# Autodesk Inventor assembly: ASY MSC 400 Accsess hatch
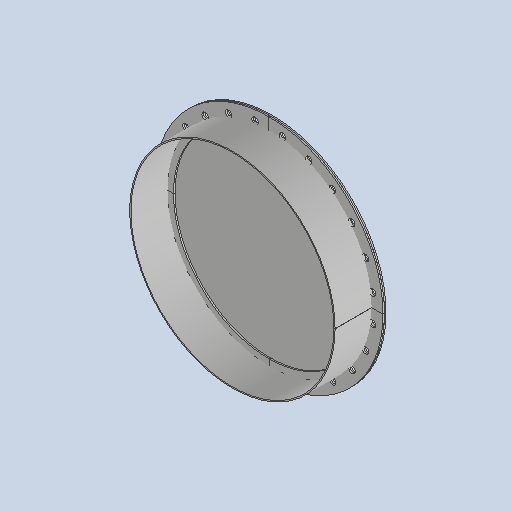
[picture p0: Inventor's stored thumbnail of the model, 512x512]
Saved by Autodesk Inventor 2025 (Build 290162010, 162A)
## iProperties
Created: 2024-09-04
Part Number: ASY MSC 400 Accsess hatch
Document SubType Name: Assembly
Designer: admin
Stock Number: ASY МОО 400 люк доступа
Author: admin
## Documents named in this file (6)
- C:\Users\DELL\YandexDisk-badmisterfox\домашниий пк\Inventor\Manturovo\Manturovo_Se-clar\ASY MSC 400 Accsess hatch.iam
- C:\Users\DELL\YandexDisk-badmisterfox\домашниий пк\Inventor\Manturovo\Manturovo_Se-clar\MSC 402 ring.ipt
- C:\Users\DELL\YandexDisk-badmisterfox\домашниий пк\Inventor\Manturovo\Manturovo_Se-clar\MSC 403 flange 500.ipt
- C:\Users\DELL\YandexDisk-badmisterfox\домашниий пк\Inventor\Manturovo\Manturovo_Se-clar\MSC 404 flange cover 500.ipt
- C:\Users\DELL\YandexDisk-badmisterfox\домашниий пк\Inventor\Manturovo\Manturovo_Se-clar\MSC 405 flange cover ring 500.ipt
- C:\Users\DELL\YandexDisk-badmisterfox\домашниий пк\Inventor\Manturovo\Manturovo_Se-clar\MSC 406 flange cover plate 500.ipt
## Components (19 placed, 5 different names)
1. MSC 402 ring:1
2. MSC 403 flange 500:1
3. MSC 403 flange 500:2
4. MSC 403 flange 500:3
5. MSC 403 flange 500:4
6. MSC 404 flange cover 500:1
7. MSC 405 flange cover ring 500:1
8. MSC 406 flange cover plate 500:1
9. MSC 406 flange cover plate 500:2
10. MSC 406 flange cover plate 500:3
11. MSC 406 flange cover plate 500:4
12. MSC 406 flange cover plate 500:5
13. MSC 406 flange cover plate 500:6
14. MSC 406 flange cover plate 500:7
15. MSC 406 flange cover plate 500:8
16. MSC 406 flange cover plate 500:9
17. MSC 406 flange cover plate 500:10
18. MSC 406 flange cover plate 500:11
19. MSC 406 flange cover plate 500:12
## Component patterns: (12 elements, first: MSC 406 flange cover plate 500:1)
## Relationships (10: WeldJoint 5, Mate 3, RevoluteJoint 1, Tangent 1)
- [WeldJoint]: MSC 403 flange 500:1 ↔ MSC 403 flange 500:2
- [WeldJoint]: MSC 403 flange 500:2 ↔ MSC 403 flange 500:3
- [WeldJoint]: MSC 403 flange 500:3 ↔ MSC 403 flange 500:4
- [RevoluteJoint]: MSC 403 flange 500:4 ↔ MSC 404 flange cover 500:1
- [Mate]: MSC 403 flange 500:3 ↔ MSC 404 flange cover 500:1
- [WeldJoint]: MSC 404 flange cover 500:1 ↔ MSC 405 flange cover ring 500:1
- [Mate]: MSC 404 flange cover 500:1 ↔ MSC 406 flange cover plate 500:1
- [Mate]: MSC 405 flange cover ring 500:1 ↔ MSC 406 flange cover plate 500:1
- [Tangent]: MSC 405 flange cover ring 500:1 ↔ MSC 406 flange cover plate 500:1
- [WeldJoint]: MSC 402 ring:1 ↔ MSC 403 flange 500:2
